# Autodesk Inventor assembly: Manipulo
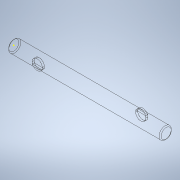
[picture p0: Inventor's stored thumbnail of the model, 180x180]
Saved by Autodesk Inventor 2021 (Build 250183000, 183)
## iProperties
Created: 2022-03-08
Part Number: Manipulo
Document SubType Name: Assembly
Designer: aluno
Author: aluno
## Documents named in this file (3)
- E:\SENAI\Terceiro semestre\TPMC - Tecnololgia de produção mecatrônica\Grampo paralelo\Manipulo.iam
- E:\SENAI\Terceiro semestre\TPMC - Tecnololgia de produção mecatrônica\Grampo paralelo\Mainpulo.ipt
- E:\SENAI\Terceiro semestre\TPMC - Tecnololgia de produção mecatrônica\Grampo paralelo\Trava.ipt
## Components (3 placed, 2 different names)
1. Mainpulo:1 — Coincidente:1, Tangente:1, Coincidente:2, Tangente:2
2. Trava:1 — Coincidente:1, Tangente:1
3. Trava:2 — Coincidente:2, Tangente:2
## Relationships (4: Mate 2, Tangent 2)
- Coincidente:1 [Mate]: Mainpulo:1 ↔ Trava:1
- Tangente:1: Mainpulo:1 ↔ Trava:1
- Coincidente:2 [Mate]: Mainpulo:1 ↔ Trava:2
- Tangente:2: Mainpulo:1 ↔ Trava:2
